# Autodesk Inventor assembly: ensamble_general
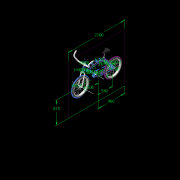
[picture p0: Inventor's stored thumbnail of the model, 180x180]
Saved by Autodesk Inventor 2021 (Build 250183000, 183)
## iProperties
Created: 2021-04-10
Part Number: ensamble_general
Document SubType Name: Assembly
Designer: j2seb
Author: j2seb
## Documents named in this file (8)
- C:\Users\maaro\Documents\UNAL\Automatización de Procesos de Manufactura\Github\Proyecto_APM\02 Inventor\ensamble_general.iam
- C:\Users\maaro\Documents\UNAL\Automatización de Procesos de Manufactura\Github\Proyecto_APM\02 Inventor\Marco_Bicicleta.iam
- C:\Users\maaro\Documents\UNAL\Automatización de Procesos de Manufactura\Github\Proyecto_APM\02 Inventor\Manubrio.ipt
- C:\Users\maaro\Documents\UNAL\Automatización de Procesos de Manufactura\Github\Proyecto_APM\02 Inventor\Ensamble_Llanta.iam
- C:\Users\maaro\Documents\UNAL\Automatización de Procesos de Manufactura\Github\Proyecto_APM\02 Inventor\sillin.iam
- C:\Users\maaro\Documents\UNAL\Automatización de Procesos de Manufactura\Github\Proyecto_APM\02 Inventor\Transmision\Design Accelerator\Roller Chain Sprocket11.ipt
- C:\Users\maaro\Documents\UNAL\Automatización de Procesos de Manufactura\Github\Proyecto_APM\02 Inventor\Transmision\Design Accelerator\Roller Chain Sprocket21.ipt
- C:\Users\maaro\Documents\UNAL\Automatización de Procesos de Manufactura\Github\Proyecto_APM\02 Inventor\Transmision\Cadena.iam
## Components (8 placed, 7 different names)
1. Marco_Bicicleta:1 [sub-assembly] — Coincidencia:2, Coincidencia:3, Flush:1, Cylindrical:2, Mate:5, Mate:6, Mate:8, Mate:10
2. Manubrio:1 — Flush:1, Cylindrical:3, Mate:7, Mate:8
3. Ensamble_Llanta:1 [sub-assembly] — Coincidencia:2
4. Ensamble_Llanta:2 [sub-assembly] — Cylindrical:3
5. sillin:1 [sub-assembly] — Cylindrical:2, Mate:5
6. Roller Chain Sprocket1:1 — Mate:14, Mate:18
7. Roller Chain Sprocket2:1 — Mate:13, Mate:16, Mate:17
8. Cadena:1 [sub-assembly] — Mate:15, Mate:16, Mate:18
## Relationships (17: Mate 13, CylindricalJoint 2, Angle 1, Flush 1)
- Coincidencia:2 [Mate]: Marco_Bicicleta:1 ↔ Ensamble_Llanta:1
- Coincidencia:3 [Mate]: Marco_Bicicleta:1
- Ángulo:1 [Angle] (0 deg)
- Flush:1 (-55.052 mm): Marco_Bicicleta:1 ↔ Manubrio:1
- Cylindrical:2: Marco_Bicicleta:1 ↔ sillin:1
- Mate:5 (-50 mm): Marco_Bicicleta:1 ↔ sillin:1
- Cylindrical:3: Manubrio:1 ↔ Ensamble_Llanta:2
- Mate:6: Marco_Bicicleta:1
- Mate:7: Manubrio:1
- Mate:8: Marco_Bicicleta:1 ↔ Manubrio:1
- Mate:10: Marco_Bicicleta:1
- Mate:13: Roller Chain Sprocket2:1
- Mate:14: Roller Chain Sprocket1:1
- Mate:15: Cadena:1
- Mate:16: Roller Chain Sprocket2:1 ↔ Cadena:1
- Mate:17: Roller Chain Sprocket2:1
- Mate:18: Roller Chain Sprocket1:1 ↔ Cadena:1
## Named parameters: DExtTub = 42.164 mm, DintTub = 35.052 mm, DIntTubTen = 28 mm, DAguUniMarcoLlanta = 4 mm
